# Autodesk Inventor assembly: Pulley with limit plates
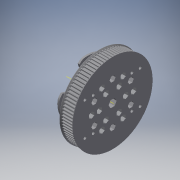
[picture p0: Inventor's stored thumbnail of the model, 180x180]
Saved by Autodesk Inventor 2018.3 (Build 223284000, 284)
## iProperties
Created: 2019-09-02
Part Number: Pulley with limit plates
Document SubType Name: Assembly
Designer: Srinity
Author: Srinity
## Documents named in this file (3)
- C:\Users\Srinity\Documents\DIY Projects\NerfGun\Pulley with limit plates.iam
- C:\Users\Srinity\Documents\DIY Projects\NerfGun\45814-B.ipt
- C:\Users\Srinity\Documents\DIY Projects\NerfGun\RotateLimitPlate.ipt
## Components (3 placed, 2 different names)
1. 45814-B:1 — Insert:1, Insert:2
2. RotateLimitPlate:1 — Insert:1, Insert:2, Insert:3, Insert:4
3. RotateLimitPlate:2 — Insert:3, Insert:4
## Relationships (4: Insert 4)
- Insert:1: 45814-B:1 ↔ RotateLimitPlate:1
- Insert:2: 45814-B:1 ↔ RotateLimitPlate:1
- Insert:3: RotateLimitPlate:1 ↔ RotateLimitPlate:2
- Insert:4: RotateLimitPlate:1 ↔ RotateLimitPlate:2
